# Autodesk Inventor assembly: Pull Tester
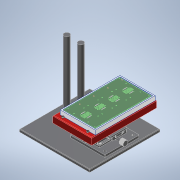
[picture p0: Inventor's stored thumbnail of the model, 180x180]
Saved by Autodesk Inventor 2022 (Build 260153000, 153)
## iProperties
Created: 2020-11-12
Part Number: Pull Tester
Document SubType Name: Assembly
Designer: caleb
Author: caleb
## Documents named in this file (8)
- C:\Users\Caleb\Desktop\nebraska-silicon-lab\Hardware\Pull Tester\Pull Tester.iam
- C:\Users\Caleb\Desktop\nebraska-silicon-lab\Hardware\Pull Tester\Chuck.ipt
- C:\Users\Caleb\Desktop\nebraska-silicon-lab\Hardware\Pull Tester\90128A211_ZNC-PLTD ALLOY STL SCKT HEAD CAP SCREW.ipt
- C:\Users\Caleb\Desktop\nebraska-silicon-lab\Hardware\Pull Tester\step_12694.ipt
- C:\Users\Caleb\Desktop\nebraska-silicon-lab\Hardware\Pull Tester\FTK100.ipt
- C:\Users\Caleb\Desktop\nebraska-silicon-lab\Hardware\ETL\Module Assembly\Tamale Assembly Plate V2\Tamale Assembly Plate 0p625in with PCB.iam
- C:\Users\Caleb\Desktop\nebraska-silicon-lab\Hardware\Pull Tester\92871A269_18-8 Stainless Steel Unthreaded Spacer.ipt
- C:\Users\Caleb\Desktop\nebraska-silicon-lab\Hardware\Pull Tester\91290A184_Black-Oxide Alloy Steel Socket Head Screw.ipt
## Components (16 placed, 7 different names)
1. Chuck:1 — Insert:22, Insert:23, Insert:24, Angle:4, Angle:6, Insert:32, Mate:4, Mate:5, Insert:37, Insert:38, Insert:39, Insert:40, Insert:41
2. 90128A211_ZNC-PLTD ALLOY STL SCKT HEAD CAP SCREW:1 — Insert:24
3. 90128A211_ZNC-PLTD ALLOY STL SCKT HEAD CAP SCREW:2 — Insert:23
4. 90128A211_ZNC-PLTD ALLOY STL SCKT HEAD CAP SCREW:3 — Insert:22
5. step_12694:1 — Mate:2, Angle:2, Flush:1, Flush:2, Insert:33, Insert:34, Insert:35, Insert:36
6. FTK100:1 — Mate:2, Angle:2, Flush:1, Flush:2, Angle:4, Angle:6
7. 90128A211_ZNC-PLTD ALLOY STL SCKT HEAD CAP SCREW:4 — Insert:32
8. Tamale Assembly Plate 0p625in with PCB:1 [sub-assembly] — Mate:4
9. 92871A269_18-8 Stainless Steel Unthreaded Spacer:1 — Insert:35
10. 92871A269_18-8 Stainless Steel Unthreaded Spacer:2 — Insert:34, Mate:5
11. 92871A269_18-8 Stainless Steel Unthreaded Spacer:3 — Insert:36, Insert:37
12. 92871A269_18-8 Stainless Steel Unthreaded Spacer:4 — Insert:33
13. 91290A184_Black-Oxide Alloy Steel Socket Head Screw:1 — Insert:38
14. 91290A184_Black-Oxide Alloy Steel Socket Head Screw:2 — Insert:39
15. 91290A184_Black-Oxide Alloy Steel Socket Head Screw:3 — Insert:40
16. 91290A184_Black-Oxide Alloy Steel Socket Head Screw:4 — Insert:41
## Relationships (21: Insert 13, Mate 3, Angle 3, Flush 2)
- Insert:22: Chuck:1 ↔ 90128A211_ZNC-PLTD ALLOY STL SCKT HEAD CAP SCREW:3
- Insert:23: Chuck:1 ↔ 90128A211_ZNC-PLTD ALLOY STL SCKT HEAD CAP SCREW:2
- Insert:24: Chuck:1 ↔ 90128A211_ZNC-PLTD ALLOY STL SCKT HEAD CAP SCREW:1
- Mate:2: step_12694:1 ↔ FTK100:1
- Angle:2 (0 deg): step_12694:1 ↔ FTK100:1
- Flush:1 (-10.16 mm): step_12694:1 ↔ FTK100:1
- Flush:2 (64.77 mm): step_12694:1 ↔ FTK100:1
- Angle:4 (0 deg): Chuck:1 ↔ FTK100:1
- Angle:6 (0 deg): Chuck:1 ↔ FTK100:1
- Insert:32: Chuck:1 ↔ 90128A211_ZNC-PLTD ALLOY STL SCKT HEAD CAP SCREW:4
- Mate:4: Chuck:1 ↔ Tamale Assembly Plate 0p625in with PCB:1
- Insert:33: step_12694:1 ↔ 92871A269_18-8 Stainless Steel Unthreaded Spacer:4
- Insert:34: step_12694:1 ↔ 92871A269_18-8 Stainless Steel Unthreaded Spacer:2
- Insert:35: step_12694:1 ↔ 92871A269_18-8 Stainless Steel Unthreaded Spacer:1
- Insert:36: step_12694:1 ↔ 92871A269_18-8 Stainless Steel Unthreaded Spacer:3
- Mate:5: Chuck:1 ↔ 92871A269_18-8 Stainless Steel Unthreaded Spacer:2
- Insert:37: Chuck:1 ↔ 92871A269_18-8 Stainless Steel Unthreaded Spacer:3
- Insert:38: Chuck:1 ↔ 91290A184_Black-Oxide Alloy Steel Socket Head Screw:1
- Insert:39: Chuck:1 ↔ 91290A184_Black-Oxide Alloy Steel Socket Head Screw:2
- Insert:40: Chuck:1 ↔ 91290A184_Black-Oxide Alloy Steel Socket Head Screw:3
- Insert:41: Chuck:1 ↔ 91290A184_Black-Oxide Alloy Steel Socket Head Screw:4
